# Autodesk Inventor assembly: two_wheels
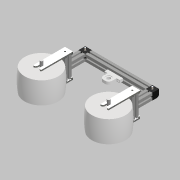
[picture p0: Inventor's stored thumbnail of the model, 180x180]
Saved by Autodesk Inventor 2021.2 (Build 252289000, 289)
## iProperties
Created: 2021-05-27
Part Number: two_wheels
Document SubType Name: Assembly
Designer: gisen
Author: gisen
## Documents named in this file (6)
- C:\Users\gisen\workspace\beetle_inventor_model\suspension\bogie.iam
- C:\Users\gisen\workspace\beetle_inventor_model\suspension\wheel_with_mounts.iam
- C:\Users\gisen\workspace\beetle_inventor_model\suspension\C-BGHKA6902ZZ-30\C-BGHKA6902ZZ-30.iam
- C:\Users\gisen\workspace\beetle_inventor_model\suspension\frame\AFS-3030-60.ipt
- C:\Users\gisen\workspace\beetle_inventor_model\suspension\frame\AFS-3030-270.ipt
- C:\Users\gisen\workspace\beetle_inventor_model\suspension\frame\ABC-3030-6.ipt
## Components (8 placed, 5 different names)
1. wheel_with_mounts:1 [sub-assembly] — メイト:18, フラッシュ:19, メイト:33, フラッシュ:38, メイト:48
2. C-BGHKA6902ZZ-30:1 [sub-assembly] — メイト:38, メイト:39, メイト:40, メイト:41
3. AFS-3030-60:1 — フラッシュ:24, メイト:27, フラッシュ:25, フラッシュ:26, メイト:42, フラッシュ:37, メイト:37, メイト:47, 対称度:1, メイト:43
4. AFS-3030-60:2 — フラッシュ:24, メイト:28, フラッシュ:25, メイト:33, 対称度:1, メイト:45, フラッシュ:38, メイト:48
5. AFS-3030-270:1 — メイト:27, メイト:28, フラッシュ:26, メイト:42, メイト:38, メイト:39, メイト:40, メイト:44, メイト:46
6. wheel_with_mounts:2 [sub-assembly] — フラッシュ:37, メイト:37, メイト:47, フラッシュ:31
7. ABC-3030-6:1 — メイト:43, メイト:44
8. ABC-3030-6:2 — メイト:45, メイト:46
## Relationships (30: Mate 22, Flush 7, Symmetry 1)
- メイト:10 [Mate]
- メイト:11 [Mate]
- メイト:12 [Mate]
- メイト:13 [Mate]
- メイト:14 [Mate] (200 mm)
- メイト:16 [Mate]
- メイト:18 [Mate]: wheel_with_mounts:1
- フラッシュ:19 [Flush]: wheel_with_mounts:1
- フラッシュ:24 [Flush]: AFS-3030-60:1 ↔ AFS-3030-60:2
- メイト:27 [Mate]: AFS-3030-60:1 ↔ AFS-3030-270:1
- メイト:28 [Mate]: AFS-3030-60:2 ↔ AFS-3030-270:1
- フラッシュ:25 [Flush]: AFS-3030-60:1 ↔ AFS-3030-60:2
- フラッシュ:26 [Flush]: AFS-3030-60:1 ↔ AFS-3030-270:1
- メイト:42 [Mate]: AFS-3030-60:1 ↔ AFS-3030-270:1
- メイト:33 [Mate]: wheel_with_mounts:1 ↔ AFS-3030-60:2
- フラッシュ:37 [Flush]: AFS-3030-60:1 ↔ wheel_with_mounts:2
- メイト:37 [Mate]: AFS-3030-60:1 ↔ wheel_with_mounts:2
- メイト:47 [Mate] (33.5 mm): AFS-3030-60:1 ↔ wheel_with_mounts:2
- 対称度:1 [Symmetry]: AFS-3030-60:1 ↔ AFS-3030-60:2
- メイト:38 [Mate]: C-BGHKA6902ZZ-30:1 ↔ AFS-3030-270:1
- メイト:39 [Mate] (-15 mm): C-BGHKA6902ZZ-30:1 ↔ AFS-3030-270:1
- メイト:40 [Mate] (-15 mm): C-BGHKA6902ZZ-30:1 ↔ AFS-3030-270:1
- メイト:41 [Mate]: C-BGHKA6902ZZ-30:1
- フラッシュ:31 [Flush]: wheel_with_mounts:2
- メイト:43 [Mate]: AFS-3030-60:1 ↔ ABC-3030-6:1
- メイト:44 [Mate]: AFS-3030-270:1 ↔ ABC-3030-6:1
- メイト:45 [Mate]: AFS-3030-60:2 ↔ ABC-3030-6:2
- メイト:46 [Mate]: AFS-3030-270:1 ↔ ABC-3030-6:2
- フラッシュ:38 [Flush]: wheel_with_mounts:1 ↔ AFS-3030-60:2
- メイト:48 [Mate] (33.5 mm): wheel_with_mounts:1 ↔ AFS-3030-60:2
